# Autodesk Inventor assembly: Electrical Board B
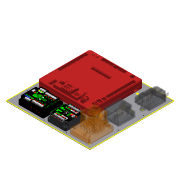
[picture p0: Inventor's stored thumbnail of the model, 180x180]
Saved by Autodesk Inventor 2015 (Build 190159000, 159)
## iProperties
Created: 2015-01-12
Part Number: Electrical Board B
Document SubType Name: Assembly
Designer: Peter
Author: Peter
## Documents named in this file (7)
- C:\Users\Tanner\Documents\GitHub\FIRST-Team-1719-CAD-Team\2015 Robot CAD\Electrical\Electrical Board B.iam
- C:\Users\Tanner\Documents\GitHub\FIRST-Team-1719-CAD-Team\2015 Robot CAD\Imported Components\Spike.ipt
- C:\Users\Tanner\Documents\GitHub\FIRST-Team-1719-CAD-Team\2015 Robot CAD\Imported Components\Victor 888 Motor Controller.ipt
- C:\Users\Tanner\Documents\GitHub\FIRST-Team-1719-CAD-Team\2015 Robot CAD\Imported Components\Pneumatics Control Module 2015.ipt
- C:\Users\Tanner\Documents\GitHub\FIRST-Team-1719-CAD-Team\2015 Robot CAD\Imported Components\Voltage Regulator Module - 2015.ipt
- C:\Users\Tanner\Documents\GitHub\FIRST-Team-1719-CAD-Team\2015 Robot CAD\Imported Components\RoboRIO.ipt
- C:\Users\Tanner\Documents\GitHub\FIRST-Team-1719-CAD-Team\2015 Robot CAD\Electrical\Power Board - Plate B.ipt
## Components (7 placed, 6 different names)
1. Spike:1 — Mate:13, Mate:14, Mate:15
2. Victor 888 Motor Controller:1 — Mate:10, Mate:11, Mate:12
3. Pneumatics Control Module 2015:1 — Mate:4, Mate:5, Mate:6
4. Voltage Regulator Module - 2015:1 — Mate:7, Mate:8, Mate:9
5. Power Board - Plate B:1 — Mate:1, Mate:2, Mate:3, Mate:4, Mate:5, Mate:6, Mate:7, Mate:8, Mate:9, Mate:10, Mate:11, Mate:12, Mate:13, Mate:14, Mate:15, Mate:16, Mate:17, Mate:18
6. RoboRIO:2 — Mate:1, Mate:2, Mate:3
7. Spike:2 — Mate:16, Mate:17, Mate:18
## Relationships (18: Mate 18)
- Mate:1: Power Board - Plate B:1 ↔ RoboRIO:2
- Mate:2 (12.7 mm): Power Board - Plate B:1 ↔ RoboRIO:2
- Mate:3 (12.7 mm): Power Board - Plate B:1 ↔ RoboRIO:2
- Mate:4: Pneumatics Control Module 2015:1 ↔ Power Board - Plate B:1
- Mate:5: Pneumatics Control Module 2015:1 ↔ Power Board - Plate B:1
- Mate:6: Pneumatics Control Module 2015:1 ↔ Power Board - Plate B:1
- Mate:7: Voltage Regulator Module - 2015:1 ↔ Power Board - Plate B:1
- Mate:8: Voltage Regulator Module - 2015:1 ↔ Power Board - Plate B:1
- Mate:9: Voltage Regulator Module - 2015:1 ↔ Power Board - Plate B:1
- Mate:10: Victor 888 Motor Controller:1 ↔ Power Board - Plate B:1
- Mate:11: Victor 888 Motor Controller:1 ↔ Power Board - Plate B:1
- Mate:12: Victor 888 Motor Controller:1 ↔ Power Board - Plate B:1
- Mate:13: Spike:1 ↔ Power Board - Plate B:1
- Mate:14: Spike:1 ↔ Power Board - Plate B:1
- Mate:15: Spike:1 ↔ Power Board - Plate B:1
- Mate:16: Power Board - Plate B:1 ↔ Spike:2
- Mate:17: Power Board - Plate B:1 ↔ Spike:2
- Mate:18: Power Board - Plate B:1 ↔ Spike:2
